# Autodesk Inventor assembly: Assembly3
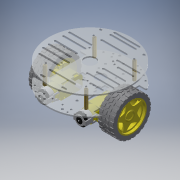
[picture p0: Inventor's stored thumbnail of the model, 180x180]
Saved by Autodesk Inventor 2019 (Build 230136000, 136)
## iProperties
Created: 2023-05-02
Part Number: Assembly3
Document SubType Name: Assembly
Designer: Tecneu Technology
Author: Tecneu Technology
## Documents named in this file (6)
- C:\Users\Tecneu Technology\TECNEU TECHNOLOGY\Tecneu Team - Documentos\Migue_2023\Modelos 3D\Chasis Carro circular Arduino\Assembly3.iam
- C:\Users\Tecneu Technology\TECNEU TECHNOLOGY\Tecneu Team - Documentos\Migue_2023\Modelos 3D\Chasis Carro circular Arduino\Part2_Estructura pequeña.ipt
- C:\Users\Tecneu Technology\TECNEU TECHNOLOGY\Tecneu Team - Documentos\Migue_2023\Modelos 3D\Chasis Carro circular Arduino\Part3_Poste largo de latón.ipt
- C:\Users\Tecneu Technology\TECNEU TECHNOLOGY\Tecneu Team - Documentos\Migue_2023\Modelos 3D\Chasis Carro circular Arduino\Part1-Estructura grande.ipt
- C:\Users\Tecneu Technology\TECNEU TECHNOLOGY\Tecneu Team - Documentos\Migue_2023\Modelos 3D\Motorreductor48a1.ipt
- C:\Users\Tecneu Technology\TECNEU TECHNOLOGY\Tecneu Team - Documentos\Migue_2023\Modelos 3D\Chasis Carro circular Arduino\Ensamble de llanta v1.iam
## Components (10 placed, 5 different names)
1. Part2_Estructura pequeña:1 — Mate:1, Mate:2, Flush:1, Mate:3, Mate:4, Mate:5, Mate:6, Mate:7, Mate:8, Mate:10, Mate:11, Flush:5, Mate:12, Flush:6, Mate:13, Mate:16, Mate:17
2. Part3_Poste largo de latón:1 — Mate:6, Flush:2, Flush:3
3. Part3_Poste largo de latón:2 — Mate:5, Flush:2
4. Part3_Poste largo de latón:3 — Mate:3, Flush:4, Mate:7, Mate:9
5. Part3_Poste largo de latón:4 — Mate:4, Flush:3, Flush:4
6. Part1-Estructura grande:1 — Mate:8, Mate:9
7. Motorreductor48a1:1 — Mate:12, Flush:6, Mate:13, Mate:14
8. Motorreductor48a1:2 — Mate:10, Mate:11, Flush:5, Mate:15
9. Ensamble de llanta v1:1 [sub-assembly] — Mate:14, Mate:16
10. Ensamble de llanta v1:2 [sub-assembly] — Mate:15, Mate:17
## Relationships (23: Mate 17, Flush 6)
- Mate:1: Part2_Estructura pequeña:1
- Mate:2: Part2_Estructura pequeña:1
- Flush:1: Part2_Estructura pequeña:1
- Mate:3: Part2_Estructura pequeña:1 ↔ Part3_Poste largo de latón:3
- Mate:4: Part2_Estructura pequeña:1 ↔ Part3_Poste largo de latón:4
- Mate:5: Part2_Estructura pequeña:1 ↔ Part3_Poste largo de latón:2
- Mate:6: Part2_Estructura pequeña:1 ↔ Part3_Poste largo de latón:1
- Flush:2: Part3_Poste largo de latón:1 ↔ Part3_Poste largo de latón:2
- Flush:3: Part3_Poste largo de latón:1 ↔ Part3_Poste largo de latón:4
- Flush:4: Part3_Poste largo de latón:3 ↔ Part3_Poste largo de latón:4
- Mate:7: Part2_Estructura pequeña:1 ↔ Part3_Poste largo de latón:3
- Mate:8: Part2_Estructura pequeña:1 ↔ Part1-Estructura grande:1
- Mate:9: Part3_Poste largo de latón:3 ↔ Part1-Estructura grande:1
- Mate:10: Part2_Estructura pequeña:1 ↔ Motorreductor48a1:2
- Mate:11: Part2_Estructura pequeña:1 ↔ Motorreductor48a1:2
- Flush:5: Part2_Estructura pequeña:1 ↔ Motorreductor48a1:2
- Mate:12: Part2_Estructura pequeña:1 ↔ Motorreductor48a1:1
- Flush:6: Part2_Estructura pequeña:1 ↔ Motorreductor48a1:1
- Mate:13: Part2_Estructura pequeña:1 ↔ Motorreductor48a1:1
- Mate:14: Motorreductor48a1:1 ↔ Ensamble de llanta v1:1
- Mate:15: Motorreductor48a1:2 ↔ Ensamble de llanta v1:2
- Mate:16 (1 mm): Part2_Estructura pequeña:1 ↔ Ensamble de llanta v1:1
- Mate:17 (1 mm): Part2_Estructura pequeña:1 ↔ Ensamble de llanta v1:2
